# Autodesk Inventor assembly: CellWithFlowDirector
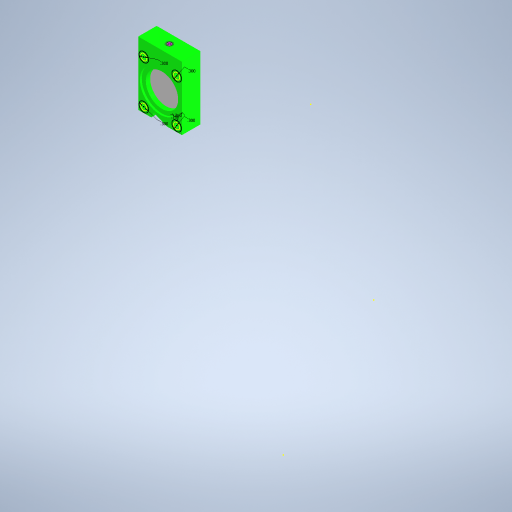
[picture p0: Inventor's stored thumbnail of the model, 512x512]
Saved by Autodesk Inventor 2024.1 (Build 281209000, 209)
## iProperties
Created: 2024-08-24
Part Number: CellWithFlowDirector
Document SubType Name: Assembly
Designer: pab2
Author: pab2
## Documents named in this file (3)
- C:\Users\pab2\Documents\GitHub\AFL-hardware-devel\Instrument-Interfacing\NCNR SANS\CellWithFlowDirector.iam
- C:\Users\pab2\Documents\GitHub\AFL-hardware-devel\Instrument-Interfacing\NCNR SANS\2 mm Ti cell - for resin printing.ipt
- C:\Users\pab2\Documents\GitHub\AFL-hardware-devel\Instrument-Interfacing\NCNR SANS\flow director r1.ipt
## Components (2 placed, 2 different names)
1. 2 mm Ti cell - for resin printing:1 — Mate:1, Mate:2
2. flow director r1:1 — Mate:1, Mate:2
## Relationships (2: Mate 2)
- Mate:1: 2 mm Ti cell - for resin printing:1 ↔ flow director r1:1
- Mate:2: 2 mm Ti cell - for resin printing:1 ↔ flow director r1:1
